# Autodesk Inventor assembly: shaft_assembly
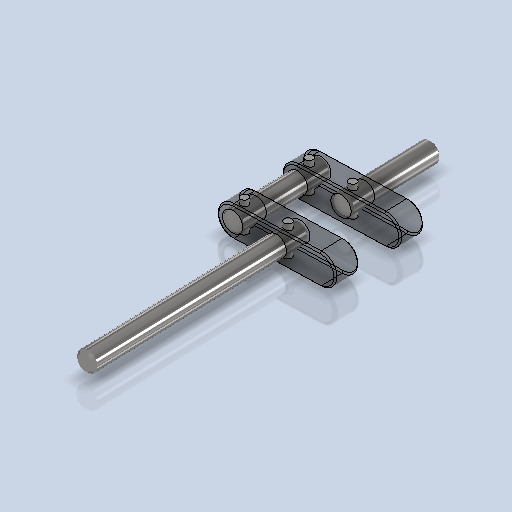
[picture p0: Inventor's stored thumbnail of the model, 512x512]
Saved by Autodesk Inventor 2024.2 (Build 282272000, 272)
## iProperties
Created: 2024-05-14
Part Number: shaft_assembly
Document SubType Name: Assembly
Designer: Fabri
Author: Fabri
## Documents named in this file (6)
- C:\Users\Fabri\Documents\Inventor\Stirlingfan\shaft_assembly.iam
- C:\Users\Fabri\Documents\Inventor\Stirlingfan\BMS_support.ipt
- C:\Users\Fabri\Documents\Inventor\Stirlingfan\BMS_bolts.ipt
- C:\Users\Fabri\Documents\Inventor\Stirlingfan\BMS_bolt_small.ipt
- C:\Users\Fabri\Documents\Inventor\Stirlingfan\BMS_fiiting_long.ipt
- C:\Users\Fabri\Documents\Inventor\Stirlingfan\BMS_bolts_left.ipt
## Components (9 placed, 5 different names)
1. BMS_support:1 — Einfügen:6, Winkel:1, Drehbar:2, Drehbar:4, Zylindrisch:2
2. BMS_support:2 — Einfügen:5, Winkel:1, Drehbar:3, Drehbar:5, Zylindrisch:1
3. BMS_bolt_small:1 — Drehbar:2
4. BMS_bolt_small:2 — Drehbar:3
5. BMS_fiiting_long:1 — Zylindrisch:1
6. BMS_bolts:2 — Zylindrisch:2
7. BMS_bolts_left:1 — Einfügen:5, Einfügen:6
8. BMS_bolt_small:3 — Drehbar:5
9. BMS_bolt_small:4 — Drehbar:4
## Relationships (9: RevoluteJoint 4, Insert 2, CylindricalJoint 2, Angle 1)
- Einfügen:5 [Insert] (-8 mm): BMS_support:2 ↔ BMS_bolts_left:1
- Einfügen:6 [Insert] (-8 mm): BMS_support:1 ↔ BMS_bolts_left:1
- Winkel:1 [Angle] (0 deg): BMS_support:1 ↔ BMS_support:2
- Drehbar:2 [RevoluteJoint] (-10 mm): BMS_support:1 ↔ BMS_bolt_small:1
- Drehbar:3 [RevoluteJoint] (10 mm): BMS_support:2 ↔ BMS_bolt_small:2
- Drehbar:4 [RevoluteJoint] (10 mm): BMS_support:1 ↔ BMS_bolt_small:4
- Drehbar:5 [RevoluteJoint] (10 mm): BMS_support:2 ↔ BMS_bolt_small:3
- Zylindrisch:1 [CylindricalJoint]: BMS_support:2 ↔ BMS_fiiting_long:1
- Zylindrisch:2 [CylindricalJoint]: BMS_support:1 ↔ BMS_bolts:2
